# Autodesk Inventor assembly: LPS_2
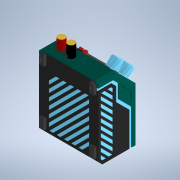
[picture p0: Inventor's stored thumbnail of the model, 180x180]
Saved by Autodesk Inventor 2022 (Build 260153000, 153)
## iProperties
Created: 2024-07-09
Part Number: LPS_2
Document SubType Name: Assembly
Designer: Капустяник Андрей
Author: Капустяник Андрей
## Documents named in this file (29)
- C:\Users\akapu\OneDrive\Документы\Git\camp2024\LPC_case\LPS_2.iam
- C:\Users\akapu\OneDrive\Документы\Git\camp2024\LPC_case\ipt\Переключатель сетевой B100G-R SWR41.ipt
- C:\Users\akapu\OneDrive\Документы\Git\camp2024\LPC_case\ipt\User Library-potenciometro.ipt
- C:\Users\akapu\OneDrive\Документы\Git\camp2024\LPC_case\ipt\volt-amp_boitier.ipt
- C:\Users\akapu\OneDrive\Документы\Git\camp2024\LPC_case\ipt\volt-amp_f2p.ipt
- C:\Users\akapu\OneDrive\Документы\Git\camp2024\LPC_case\ipt\volt-amp_f3p.ipt
- C:\Users\akapu\OneDrive\Документы\Git\camp2024\LPC_case\ipt\volt-amp_pcb.ipt
- C:\Users\akapu\OneDrive\Документы\Git\camp2024\LPC_case\ipt\led_cap.ipt
- C:\Users\akapu\OneDrive\Документы\Git\camp2024\LPC_case\ipt\LPS_base.ipt
- C:\Users\akapu\OneDrive\Документы\Git\camp2024\LPC_case\ipt\LPS_board.ipt
- C:\Users\akapu\OneDrive\Документы\Git\camp2024\LPC_case\ipt\LPS_cap.ipt
- C:\Users\akapu\OneDrive\Документы\Git\camp2024\LPC_case\ipt\power unit.ipt
- C:\Users\akapu\OneDrive\Документы\Git\camp2024\LPC_case\ipt\9.5 MM PUSH BUTTON.ipt
- C:\Users\akapu\OneDrive\Документы\Git\camp2024\LPC_case\ipt\404010 Fan v5.ipt
- C:\Users\akapu\OneDrive\Документы\Git\camp2024\LPC_case\ipt\ALSRobot-LED 8mm.ipt
- C:\Users\akapu\OneDrive\Документы\Git\camp2024\LPC_case\ipt\banana plug.ipt
- C:\Users\akapu\OneDrive\Документы\Git\camp2024\LPC_case\ipt\interlock_switch_male_wFuse v13.ipt
- C:\Users\akapu\OneDrive\Документы\Git\camp2024\LPC_case\ipt\right_line.ipt
- C:\Users\akapu\OneDrive\Документы\Git\camp2024\LPC_case\ipt\left_line.ipt
- C:\Users\akapu\OneDrive\Документы\Git\camp2024\LPC_case\ipt\leg.ipt
- C:\Users\akapu\OneDrive\Документы\Git\camp2024\LPC_case\ipt\leg2.ipt
- C:\Users\akapu\OneDrive\Документы\Git\camp2024\LPC_case\ipt\leg3.ipt
- C:\Users\akapu\OneDrive\Документы\Git\camp2024\LPC_case\ipt\LPS.ipt
- C:\Users\akapu\OneDrive\Документы\Git\camp2024\LPC_case\ipt\tablet.ipt
- C:\Users\akapu\OneDrive\Документы\Git\camp2024\LPC_case\ipt\button_tablet.ipt
- C:\Users\akapu\OneDrive\Документы\Git\camp2024\LPC_case\STL\filter1.ipt
- C:\Users\akapu\OneDrive\Документы\Git\camp2024\LPC_case\STL\filter2.ipt
- C:\Users\akapu\OneDrive\Документы\Git\camp2024\LPC_case\ipt\potention_wheel_В.ipt
- C:\Users\akapu\OneDrive\Документы\Git\camp2024\LPC_case\ipt\potention_wheel_A.ipt
## Components (31 placed, 28 different names)
1. Переключатель сетевой B100G-R SWR41:1 — Совмещение:35, Совмещение:41, Совмещение:44
2. User Library-potenciometro:1 — Совмещение:34, Совмещение:46, Совмещение:56, Совмещение:59, Совмещение:61
3. volt-amp_boitier:1 — Совмещение:1, Совмещение:2, Совмещение:3, Совмещение:31, Совмещение:42, Совмещение:43
4. volt-amp_f2p:1 — Совмещение:4, Совмещение:5, Совмещение:6
5. volt-amp_f3p:1 — Совмещение:7, Совмещение:8, Совмещение:9
6. volt-amp_pcb:1 — Совмещение:1, Совмещение:2, Совмещение:3, Совмещение:4, Совмещение:5, Совмещение:6, Совмещение:7, Совмещение:8, Совмещение:9
7. LPS_base:1 — Совмещение:10, Совмещение:11, Совмещение:12, Заподлицо:1, Заподлицо:2, Совмещение:13, Совмещение:14, Совмещение:16, Совмещение:17, Совмещение:18, Совмещение:19, Заподлицо:3, Совмещение:20, Совмещение:21, Совмещение:24, Совмещение:26, Совмещение:28, Совмещение:29, Совмещение:30, Заподлицо:8, Заподлицо:9, Заподлицо:10, Заподлицо:11, Совмещение:49, Совмещение:50, Совмещение:51, Заподлицо:17, Заподлицо:18, Совмещение:57
8. LPS_board:1 — Совмещение:13, Совмещение:14, Совмещение:15, Заподлицо:13, Совмещение:37, Совмещение:38
9. LPS_cap:1 — Совмещение:30, Заподлицо:8, Заподлицо:9, Совмещение:31, Совмещение:32, Заподлицо:12, Совмещение:33, Совмещение:34, Совмещение:35, Совмещение:36, Совмещение:39, Совмещение:40, Совмещение:41, Совмещение:42, Совмещение:43, Совмещение:44, Совмещение:45, Совмещение:46, Заподлицо:14, Совмещение:47, Совмещение:48, Заподлицо:15, Совмещение:52, Совмещение:53, Совмещение:54, Совмещение:55, Совмещение:56, Заподлицо:16
10. power unit:1 — Совмещение:10, Совмещение:11, Совмещение:15, Совмещение:16
11. 9.5 MM PUSH BUTTON:1 — Совмещение:32, Совмещение:40
12. 404010 Fan v5:1 — Совмещение:17, Совмещение:18, Совмещение:19
13. ALSRobot-LED 8mm:1 — Совмещение:33, Совмещение:39
14. banana plug:1 — Заподлицо:12, Совмещение:47, Совмещение:48
15. interlock_switch_male_wFuse v13:1 — Совмещение:12, Заподлицо:1, Заподлицо:2
16. right_line:1 — Заподлицо:3
17. left_line:1 — Совмещение:20, Заподлицо:10, Заподлицо:11
18. leg:1 — Заподлицо:6, Совмещение:49, Совмещение:50
19. leg2:1 — Совмещение:21, Совмещение:24, Заподлицо:6
20. leg:2 — Совмещение:26, Заподлицо:7, Совмещение:51
21. leg3:1 — Совмещение:28, Совмещение:29, Заподлицо:7
22. User Library-potenciometro:2 — Совмещение:36, Совмещение:45, Совмещение:55, Совмещение:58, Совмещение:60
23. LPS:1 — Заподлицо:13, Совмещение:37, Совмещение:38, Заподлицо:15
24. tablet:1 — Заподлицо:14
25. led_cap:1 — Совмещение:52, Совмещение:53, Совмещение:54
26. button_tablet:1 — Заподлицо:16
27. filter1:1 — Заподлицо:17
28. filter2:1 — Заподлицо:18, Заподлицо:19, Заподлицо:20
29. filter2:2 — Заподлицо:19, Заподлицо:20, Совмещение:57
30. potention_wheel_В:1 — Совмещение:58, Совмещение:60
31. potention_wheel_A:1 — Совмещение:59, Совмещение:61
## Relationships (75: Mate 57, Flush 18)
- Совмещение:1 [Mate]: volt-amp_boitier:1 ↔ volt-amp_pcb:1
- Совмещение:2 [Mate]: volt-amp_boitier:1 ↔ volt-amp_pcb:1
- Совмещение:3 [Mate]: volt-amp_boitier:1 ↔ volt-amp_pcb:1
- Совмещение:4 [Mate]: volt-amp_f2p:1 ↔ volt-amp_pcb:1
- Совмещение:5 [Mate]: volt-amp_f2p:1 ↔ volt-amp_pcb:1
- Совмещение:6 [Mate]: volt-amp_f2p:1 ↔ volt-amp_pcb:1
- Совмещение:7 [Mate]: volt-amp_f3p:1 ↔ volt-amp_pcb:1
- Совмещение:8 [Mate]: volt-amp_f3p:1 ↔ volt-amp_pcb:1
- Совмещение:9 [Mate]: volt-amp_f3p:1 ↔ volt-amp_pcb:1
- Совмещение:10 [Mate] (4 mm): LPS_base:1 ↔ power unit:1
- Совмещение:11 [Mate] (3 mm): LPS_base:1 ↔ power unit:1
- Совмещение:12 [Mate]: LPS_base:1 ↔ interlock_switch_male_wFuse v13:1
- Заподлицо:1 [Flush] (5 mm): LPS_base:1 ↔ interlock_switch_male_wFuse v13:1
- Заподлицо:2 [Flush] (9 mm): LPS_base:1 ↔ interlock_switch_male_wFuse v13:1
- Совмещение:13 [Mate] (4 mm): LPS_base:1 ↔ LPS_board:1
- Совмещение:14 [Mate]: LPS_base:1 ↔ LPS_board:1
- Совмещение:15 [Mate] (4 mm): LPS_board:1 ↔ power unit:1
- Совмещение:16 [Mate]: LPS_base:1 ↔ power unit:1
- Совмещение:17 [Mate]: LPS_base:1 ↔ 404010 Fan v5:1
- Совмещение:18 [Mate]: LPS_base:1 ↔ 404010 Fan v5:1
- Совмещение:19 [Mate]: LPS_base:1 ↔ 404010 Fan v5:1
- Заподлицо:3 [Flush]: LPS_base:1 ↔ right_line:1
- Совмещение:20 [Mate]: LPS_base:1 ↔ left_line:1
- Совмещение:21 [Mate]: LPS_base:1 ↔ leg2:1
- Совмещение:24 [Mate]: LPS_base:1 ↔ leg2:1
- Заподлицо:6 [Flush]: leg:1 ↔ leg2:1
- Совмещение:26 [Mate]: LPS_base:1 ↔ leg:2
- Совмещение:28 [Mate]: LPS_base:1 ↔ leg3:1
- Совмещение:29 [Mate]: LPS_base:1 ↔ leg3:1
- Заподлицо:7 [Flush]: leg:2 ↔ leg3:1
- Совмещение:30 [Mate] (0.2 mm): LPS_base:1 ↔ LPS_cap:1
- Заподлицо:8 [Flush]: LPS_base:1 ↔ LPS_cap:1
- Заподлицо:9 [Flush]: LPS_base:1 ↔ LPS_cap:1
- Совмещение:31 [Mate]: volt-amp_boitier:1 ↔ LPS_cap:1
- Заподлицо:10 [Flush]: LPS_base:1 ↔ left_line:1
- Заподлицо:11 [Flush]: LPS_base:1 ↔ left_line:1
- Совмещение:32 [Mate]: LPS_cap:1 ↔ 9.5 MM PUSH BUTTON:1
- Заподлицо:12 [Flush]: LPS_cap:1 ↔ banana plug:1
- Совмещение:33 [Mate]: LPS_cap:1 ↔ ALSRobot-LED 8mm:1
- Совмещение:34 [Mate]: User Library-potenciometro:1 ↔ LPS_cap:1
- Совмещение:35 [Mate]: Переключатель сетевой B100G-R SWR41:1 ↔ LPS_cap:1
- Совмещение:36 [Mate]: LPS_cap:1 ↔ User Library-potenciometro:2
- Заподлицо:13 [Flush]: LPS_board:1 ↔ LPS:1
- Совмещение:37 [Mate]: LPS_board:1 ↔ LPS:1
- Совмещение:38 [Mate]: LPS_board:1 ↔ LPS:1
- Совмещение:39 [Mate]: LPS_cap:1 ↔ ALSRobot-LED 8mm:1
- Совмещение:40 [Mate]: LPS_cap:1 ↔ 9.5 MM PUSH BUTTON:1
- Совмещение:41 [Mate]: Переключатель сетевой B100G-R SWR41:1 ↔ LPS_cap:1
- Совмещение:42 [Mate]: volt-amp_boitier:1 ↔ LPS_cap:1
- Совмещение:43 [Mate]: volt-amp_boitier:1 ↔ LPS_cap:1
- Совмещение:44 [Mate] (1.2 mm): Переключатель сетевой B100G-R SWR41:1 ↔ LPS_cap:1
- Совмещение:45 [Mate]: LPS_cap:1 ↔ User Library-potenciometro:2
- Совмещение:46 [Mate]: User Library-potenciometro:1 ↔ LPS_cap:1
- Заподлицо:14 [Flush]: LPS_cap:1 ↔ tablet:1
- Совмещение:47 [Mate]: LPS_cap:1 ↔ banana plug:1
- Совмещение:48 [Mate]: LPS_cap:1 ↔ banana plug:1
- Заподлицо:15 [Flush]: LPS_cap:1 ↔ LPS:1
- Совмещение:49 [Mate]: LPS_base:1 ↔ leg:1
- Совмещение:50 [Mate]: LPS_base:1 ↔ leg:1
- Совмещение:51 [Mate]: LPS_base:1 ↔ leg:2
- Совмещение:52 [Mate]: LPS_cap:1 ↔ led_cap:1
- Совмещение:53 [Mate]: LPS_cap:1 ↔ led_cap:1
- Совмещение:54 [Mate]: LPS_cap:1 ↔ led_cap:1
- Совмещение:55 [Mate]: LPS_cap:1 ↔ User Library-potenciometro:2
- Совмещение:56 [Mate]: User Library-potenciometro:1 ↔ LPS_cap:1
- Заподлицо:16 [Flush]: LPS_cap:1 ↔ button_tablet:1
- Заподлицо:17 [Flush]: LPS_base:1 ↔ filter1:1
- Заподлицо:18 [Flush]: LPS_base:1 ↔ filter2:1
- Заподлицо:19 [Flush]: filter2:1 ↔ filter2:2
- Заподлицо:20 [Flush]: filter2:1 ↔ filter2:2
- Совмещение:57 [Mate]: LPS_base:1 ↔ filter2:2
- Совмещение:58 [Mate]: User Library-potenciometro:2 ↔ potention_wheel_В:1
- Совмещение:59 [Mate]: User Library-potenciometro:1 ↔ potention_wheel_A:1
- Совмещение:60 [Mate] (4 mm): User Library-potenciometro:2 ↔ potention_wheel_В:1
- Совмещение:61 [Mate] (4 mm): User Library-potenciometro:1 ↔ potention_wheel_A:1
